# Autodesk Inventor assembly: SystemAssemV2
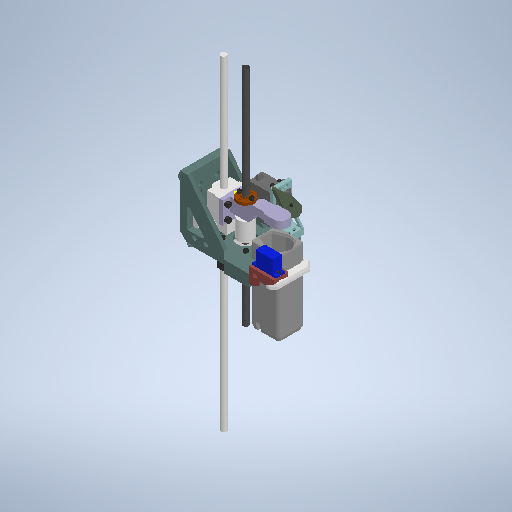
[picture p0: Inventor's stored thumbnail of the model, 512x512]
Saved by Autodesk Inventor 2025.1 (Build 291241000, 241)
## iProperties
Created: 2025-03-02
Part Number: SystemAssemV2
Document SubType Name: Assembly
Designer: 13156
Author: 13156
## Documents named in this file (25)
- C:\Users\13156\OneDrive - Binghamton University\Documents\GitHub\Perovskite-Automated-Synthesis-System\CAD\Pipette\Pippete System.iam
- C:\Users\13156\OneDrive - Binghamton University\Documents\GitHub\Perovskite-Automated-Synthesis-System\CAD\Pipette\Holder.ipt
- C:\Users\13156\OneDrive - Binghamton University\Documents\GitHub\Perovskite-Automated-Synthesis-System\CAD\Non 3D Printed Parts\Motors and Servos\NEMA17 Stepper Motor - 26 mm.ipt
- C:\Users\13156\OneDrive - Binghamton University\Documents\GitHub\Perovskite-Automated-Synthesis-System\CAD\Pipette\Pipette Sleeve.ipt
- C:\Users\13156\OneDrive - Binghamton University\Documents\GitHub\Perovskite-Automated-Synthesis-System\CAD\Non 3D Printed Parts\LeadScrewBase.ipt
- C:\Users\13156\OneDrive - Binghamton University\Documents\GitHub\Perovskite-Automated-Synthesis-System\CAD\Non 3D Printed Parts\Linear Rails\8mm Linear Rod.ipt
- C:\Users\13156\OneDrive - Binghamton University\Documents\GitHub\Perovskite-Automated-Synthesis-System\CAD\Non 3D Printed Parts\Linear Rails\Linear Bearing 8mm Square.ipt
- C:\Users\13156\OneDrive - Binghamton University\Documents\GitHub\Perovskite-Automated-Synthesis-System\CAD\Pipette\Actuator.ipt
- C:\Users\13156\OneDrive - Binghamton University\Documents\GitHub\Perovskite-Automated-Synthesis-System\CAD\Pipette\Ejector Servo Holder.ipt
- C:\Users\13156\OneDrive - Binghamton University\Documents\GitHub\Perovskite-Automated-Synthesis-System\CAD\Non 3D Printed Parts\Motors and Servos\MG 996R.ipt
- C:\Users\13156\OneDrive - Binghamton University\Documents\GitHub\Perovskite-Automated-Synthesis-System\CAD\Non 3D Printed Parts\Leadscrew.ipt
- C:\Users\13156\OneDrive - Binghamton University\Documents\GitHub\Perovskite-Automated-Synthesis-System\CAD\Pipette\Ejector Arm.ipt
- C:\Users\13156\OneDrive - Binghamton University\Documents\GitHub\Perovskite-Automated-Synthesis-System\CAD\Non 3D Printed Parts\Threaded Rod 300mm.ipt
- C:\Users\13156\OneDrive - Binghamton University\Documents\GitHub\Perovskite-Automated-Synthesis-System\CAD\Pipette\Grabber Servo Holder.ipt
- C:\Users\13156\OneDrive - Binghamton University\Documents\GitHub\Perovskite-Automated-Synthesis-System\CAD\Non 3D Printed Parts\Motors and Servos\SG90 Servo.ipt
- C:\Users\13156\OneDrive - Binghamton University\Documents\GitHub\Perovskite-Automated-Synthesis-System\CAD\Pipette\Grabber Arm.ipt
- C:\Users\13156\OneDrive - Binghamton University\Documents\GitHub\Perovskite-Automated-Synthesis-System\CAD\Non 3D Printed Parts\Motors and Servos\HalfServoArm.ipt
- C:\Users\13156\OneDrive - Binghamton University\Documents\GitHub\Perovskite-Automated-Synthesis-System\CAD\Non 3D Printed Parts\Linear Rails\Linear Rod Holder SK8.ipt
- C:\Users\13156\OneDrive - Binghamton University\Documents\GitHub\Perovskite-Automated-Synthesis-System\CAD\Non 3D Printed Parts\Screws\M4x20.ipt
- C:\Users\13156\OneDrive - Binghamton University\Documents\GitHub\Perovskite-Automated-Synthesis-System\CAD\Non 3D Printed Parts\Screws\M2x8.ipt
- C:\Users\13156\OneDrive - Binghamton University\Documents\GitHub\Perovskite-Automated-Synthesis-System\CAD\Non 3D Printed Parts\Screws\M3x6.ipt
- C:\Users\13156\OneDrive - Binghamton University\Documents\GitHub\Perovskite-Automated-Synthesis-System\CAD\Non 3D Printed Parts\Screws\M3x8.ipt
- C:\Users\13156\OneDrive - Binghamton University\Documents\GitHub\Perovskite-Automated-Synthesis-System\CAD\Non 3D Printed Parts\Nuts\M4 Nut.ipt
- C:\Users\13156\OneDrive - Binghamton University\Documents\GitHub\Perovskite-Automated-Synthesis-System\CAD\Non 3D Printed Parts\Limit Switch.ipt
- C:\Users\13156\OneDrive - Binghamton University\Documents\GitHub\Perovskite-Automated-Synthesis-System\CAD\Pipette\Pipette Stand.ipt
## Components (42 placed, 24 different names)
1. Holder:1 — Mate:1, Mate:2, Mate:3, Mate:4, Mate:5, Mate:6, Mate:7, Mate:8, Mate:9, Mate:10, Mate:13, Mate:19, Mate:20, Mate:21, Mate:26, Mate:27, Mate:28, Flush:1, Flush:3, Mate:42, Mate:43, Mate:44, Mate:52, Mate:53, Mate:54, Mate:93, Mate:94, Mate:95, Mate:96, Mate:97, Mate:98, Mate:99, Mate:100, Mate:105, Mate:106, Mate:107
2. NEMA17 Stepper Motor - 26 mm:1 — Mate:4, Mate:5, Mate:6, Mate:7, Mate:11, Mate:41
3. Pipette Sleeve:1 — Mate:8, Mate:9, Mate:10, Mate:108, Mate:109, Mate:110
4. LeadScrewBase:1 — Mate:11, Mate:40, Mate:28
5. 8mm Linear Rod:1 — Mate:13, Mate:14, Flush:1
6. Linear Bearing 8mm Square:1 — Mate:14, Mate:16, Mate:29
7. Actuator:1 — Mate:16, Mate:29, Mate:31, Mate:32, Mate:33, Mate:34, Mate:55, Mate:56, Mate:57, Mate:58, Mate:60, Mate:61, Mate:62, Mate:63
8. Ejector Servo Holder:1 — Mate:19, Mate:20, Mate:21, Mate:24, Mate:26, Mate:27, Mate:36, Mate:37, Mate:72, Mate:73, Mate:74, Mate:75, Mate:102, Mate:103
9. MG 996R:1 — Mate:24, Mate:36, Mate:37, Mate:38, Mate:39, Mate:84, Mate:85, Mate:86, Mate:87, Mate:88, Mate:89, Mate:90, Mate:91, Mate:92
10. Leadscrew:1 — Mate:31, Mate:32, Mate:33, Mate:34, Mate:40, Mate:80, Mate:81, Mate:82, Mate:83
11. Ejector Arm:1 — Mate:38, Mate:39, Mate:64, Mate:65
12. Threaded Rod 300mm:1 — Mate:41, Flush:3
13. Grabber Servo Holder:1 — Mate:42, Mate:43, Mate:44, Mate:45, Mate:46, Mate:47, Mate:68, Mate:69, Mate:70, Mate:71
14. SG90 Servo:1 — Mate:45, Mate:46, Mate:47, Mate:48, Mate:49, Mate:76, Mate:77, Mate:78, Mate:79
15. Grabber Arm:1 — Mate:50, Mate:51, Mate:59, Mate:66, Mate:67
16. HalfServoArm:1 — Mate:48, Mate:49, Mate:50, Mate:51, Mate:59
17. Linear Rod Holder SK8:1 — Mate:52, Mate:53, Mate:54
18. M4x20:1 — Mate:60, Mate:61
19. M4x20:2 — Mate:62, Mate:63
20. M4x20:3 — Mate:55, Mate:56
21. M4x20:4 — Mate:57, Mate:58
22. M2x8:4 — Mate:66, Mate:67
23. M2x8:5 — Mate:64, Mate:65
24. M2x8:6 — Mate:72, Mate:75
25. M2x8:7 — Mate:73, Mate:74
26. M2x8:8 — Mate:70, Mate:71
27. M2x8:9 — Mate:68, Mate:69
28. M2x8:11 — Mate:76, Mate:79
29. M2x8:12 — Mate:77, Mate:78
30. M3x6:1 — Mate:80, Mate:82
31. M3x6:2 — Mate:81, Mate:83
32. M3x6:3 — Mate:84, Mate:92
33. M3x6:4 — Mate:85, Mate:91
34. M3x6:5 — Mate:87, Mate:88, Mate:90
35. M3x6:6 — Mate:86, Mate:89
36. M3x8:1 — Mate:95, Mate:99
37. M3x8:2 — Mate:94, Mate:97
38. M3x8:3 — Mate:93, Mate:100
39. M3x8:4 — Mate:96, Mate:98
40. M4 Nut:1 — Mate:102, Mate:103
41. Limit Switch:1 — Mate:105, Mate:106, Mate:107
42. Pipette Stand:1 — Mate:108, Mate:109, Mate:110
## Relationships (101: Mate 99, Flush 2)
- Mate:1: Holder:1
- Mate:2: Holder:1
- Mate:3: Holder:1
- Mate:4: Holder:1 ↔ NEMA17 Stepper Motor - 26 mm:1
- Mate:5: Holder:1 ↔ NEMA17 Stepper Motor - 26 mm:1
- Mate:6: Holder:1 ↔ NEMA17 Stepper Motor - 26 mm:1
- Mate:7: Holder:1 ↔ NEMA17 Stepper Motor - 26 mm:1
- Mate:8: Holder:1 ↔ Pipette Sleeve:1
- Mate:9: Holder:1 ↔ Pipette Sleeve:1
- Mate:10: Holder:1 ↔ Pipette Sleeve:1
- Mate:11: NEMA17 Stepper Motor - 26 mm:1 ↔ LeadScrewBase:1
- Mate:13: Holder:1 ↔ 8mm Linear Rod:1
- Mate:14: 8mm Linear Rod:1 ↔ Linear Bearing 8mm Square:1
- Mate:16: Linear Bearing 8mm Square:1 ↔ Actuator:1
- Mate:19: Holder:1 ↔ Ejector Servo Holder:1
- Mate:20: Holder:1 ↔ Ejector Servo Holder:1
- Mate:21: Holder:1 ↔ Ejector Servo Holder:1
- Mate:24: Ejector Servo Holder:1 ↔ MG 996R:1
- Mate:26: Holder:1 ↔ Ejector Servo Holder:1
- Mate:27: Holder:1 ↔ Ejector Servo Holder:1
- Mate:28 (2 mm): Holder:1 ↔ LeadScrewBase:1
- Flush:1 (-200 mm): Holder:1 ↔ 8mm Linear Rod:1
- Mate:29: Linear Bearing 8mm Square:1 ↔ Actuator:1
- Mate:31: Actuator:1 ↔ Leadscrew:1
- Mate:32: Actuator:1 ↔ Leadscrew:1
- Mate:33: Actuator:1 ↔ Leadscrew:1
- Mate:34: Actuator:1 ↔ Leadscrew:1
- Mate:36: Ejector Servo Holder:1 ↔ MG 996R:1
- Mate:37 (0.5 mm): Ejector Servo Holder:1 ↔ MG 996R:1
- Mate:38: MG 996R:1 ↔ Ejector Arm:1
- Mate:39: MG 996R:1 ↔ Ejector Arm:1
- Mate:40: LeadScrewBase:1 ↔ Leadscrew:1
- Mate:41: NEMA17 Stepper Motor - 26 mm:1 ↔ Threaded Rod 300mm:1
- Flush:3 (-200 mm): Holder:1 ↔ Threaded Rod 300mm:1
- Mate:42: Holder:1 ↔ Grabber Servo Holder:1
- Mate:43: Holder:1 ↔ Grabber Servo Holder:1
- Mate:44: Holder:1 ↔ Grabber Servo Holder:1
- Mate:45: Grabber Servo Holder:1 ↔ SG90 Servo:1
- Mate:46: Grabber Servo Holder:1 ↔ SG90 Servo:1
- Mate:47: Grabber Servo Holder:1 ↔ SG90 Servo:1
- Mate:48: SG90 Servo:1 ↔ HalfServoArm:1
- Mate:49 (1 mm): SG90 Servo:1 ↔ HalfServoArm:1
- Mate:50: Grabber Arm:1 ↔ HalfServoArm:1
- Mate:51: Grabber Arm:1 ↔ HalfServoArm:1
- Mate:52: Holder:1 ↔ Linear Rod Holder SK8:1
- Mate:53: Holder:1 ↔ Linear Rod Holder SK8:1
- Mate:54: Holder:1 ↔ Linear Rod Holder SK8:1
- Mate:55: Actuator:1 ↔ M4x20:3
- Mate:56: Actuator:1 ↔ M4x20:3
- Mate:57: Actuator:1 ↔ M4x20:4
- Mate:58: Actuator:1 ↔ M4x20:4
- Mate:59: Grabber Arm:1 ↔ HalfServoArm:1
- Mate:60: Actuator:1 ↔ M4x20:1
- Mate:61: Actuator:1 ↔ M4x20:1
- Mate:62: Actuator:1 ↔ M4x20:2
- Mate:63: Actuator:1 ↔ M4x20:2
- Mate:64: Ejector Arm:1 ↔ M2x8:5
- Mate:65: Ejector Arm:1 ↔ M2x8:5
- Mate:66: Grabber Arm:1 ↔ M2x8:4
- Mate:67: Grabber Arm:1 ↔ M2x8:4
- Mate:68: Grabber Servo Holder:1 ↔ M2x8:9
- Mate:69: Grabber Servo Holder:1 ↔ M2x8:9
- Mate:70: Grabber Servo Holder:1 ↔ M2x8:8
- Mate:71: Grabber Servo Holder:1 ↔ M2x8:8
- Mate:72: Ejector Servo Holder:1 ↔ M2x8:6
- Mate:73: Ejector Servo Holder:1 ↔ M2x8:7
- Mate:74: Ejector Servo Holder:1 ↔ M2x8:7
- Mate:75: Ejector Servo Holder:1 ↔ M2x8:6
- Mate:76: SG90 Servo:1 ↔ M2x8:11
- Mate:77: SG90 Servo:1 ↔ M2x8:12
- Mate:78: SG90 Servo:1 ↔ M2x8:12
- Mate:79: SG90 Servo:1 ↔ M2x8:11
- Mate:80: Leadscrew:1 ↔ M3x6:1
- Mate:81: Leadscrew:1 ↔ M3x6:2
- Mate:82: Leadscrew:1 ↔ M3x6:1
- Mate:83: Leadscrew:1 ↔ M3x6:2
- Mate:84: MG 996R:1 ↔ M3x6:3
- Mate:85: MG 996R:1 ↔ M3x6:4
- Mate:86: MG 996R:1 ↔ M3x6:6
- Mate:87: MG 996R:1 ↔ M3x6:5
- Mate:88: MG 996R:1 ↔ M3x6:5
- Mate:89: MG 996R:1 ↔ M3x6:6
- Mate:90: MG 996R:1 ↔ M3x6:5
- Mate:91: MG 996R:1 ↔ M3x6:4
- Mate:92: MG 996R:1 ↔ M3x6:3
- Mate:93: Holder:1 ↔ M3x8:3
- Mate:94: Holder:1 ↔ M3x8:2
- Mate:95: Holder:1 ↔ M3x8:1
- Mate:96: Holder:1 ↔ M3x8:4
- Mate:97: Holder:1 ↔ M3x8:2
- Mate:98: Holder:1 ↔ M3x8:4
- Mate:99: Holder:1 ↔ M3x8:1
- Mate:100: Holder:1 ↔ M3x8:3
- Mate:102: Ejector Servo Holder:1 ↔ M4 Nut:1
- Mate:103: Ejector Servo Holder:1 ↔ M4 Nut:1
- Mate:105: Holder:1 ↔ Limit Switch:1
- Mate:106: Holder:1 ↔ Limit Switch:1
- Mate:107: Holder:1 ↔ Limit Switch:1
- Mate:108: Pipette Sleeve:1 ↔ Pipette Stand:1
- Mate:109: Pipette Sleeve:1 ↔ Pipette Stand:1
- Mate:110: Pipette Sleeve:1 ↔ Pipette Stand:1
